# Autodesk Inventor assembly: Montagem_Suporte_Rolamento_LDR
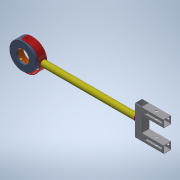
[picture p0: Inventor's stored thumbnail of the model, 180x180]
Saved by Autodesk Inventor 2022 (Build 260153000, 153)
## iProperties
Created: 2016-03-04
Part Number: Montagem_Suporte_Rolamento_LDR
Document SubType Name: Assembly
Designer: Everton
Author: Everton
## Documents named in this file (5)
- C:\Users\Alison\Documents\TCC\Peças e desenho no inventor - TCC\Peças\Montagem_Suporte_Rolamento_LDR.iam
- C:\Users\Alison\Documents\TCC\Peças e desenho no inventor - TCC\Peças\FIXADOR_APOIO_ROLAMENTO.ipt
- C:\Users\Alison\Documents\TCC\Desenhos e Montagem\desenhos e montagems inventor 15\Apoio Tubo.ipt
- C:\Users\Alison\Documents\TCC\Peças e desenho no inventor - TCC\Peças\MONTAGEM_ROLAMENTO.iam
- C:\Users\Alison\Documents\TCC\Peças e desenho no inventor - TCC\Peças\Suporte_Tubo_LDR.ipt
## Components (4 placed, 4 different names)
1. FIXADOR_APOIO_ROLAMENTO:1 — Coincidente:6, Tangente:1, Inserir:1
2. Apoio Tubo:1 — Mate:5, Coincidente:6, Tangente:1
3. MONTAGEM_ROLAMENTO:1 [sub-assembly] — Mate:5
4. Suporte_Tubo_LDR:1 — Inserir:1
## Relationships (4: Mate 2, Tangent 1, Insert 1)
- Mate:5: Apoio Tubo:1 ↔ MONTAGEM_ROLAMENTO:1
- Coincidente:6 [Mate]: FIXADOR_APOIO_ROLAMENTO:1 ↔ Apoio Tubo:1
- Tangente:1: FIXADOR_APOIO_ROLAMENTO:1 ↔ Apoio Tubo:1
- Inserir:1: FIXADOR_APOIO_ROLAMENTO:1 ↔ Suporte_Tubo_LDR:1
